# Autodesk Inventor assembly: Full_model
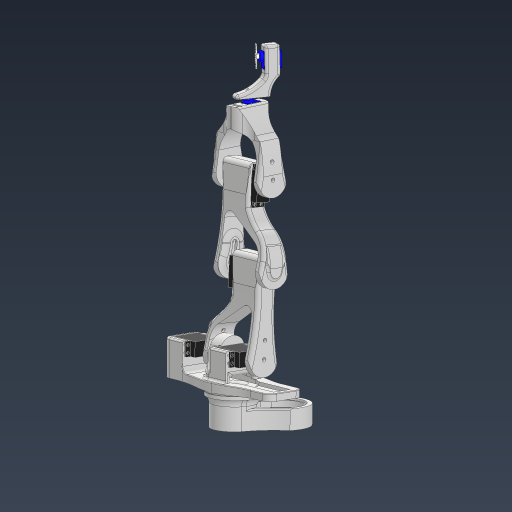
[picture p0: Inventor's stored thumbnail of the model, 512x512]
Saved by Autodesk Inventor 2024 (Build 280153000, 153)
## iProperties
Created: 2025-08-29
Part Number: Full_model
Document SubType Name: Assembly
Designer: Piter
Author: Piter
## Documents named in this file (9)
- C:\Users\Piter\OneDrive\Pulpit\Robots\david_Arm\Davie-Robot-Arm\3D Models\Full_model.iam
- C:\Users\Piter\OneDrive\Pulpit\Robots\david_Arm\Davie-Robot-Arm\3D Models\Arm2.ipt
- C:\Users\Piter\OneDrive\Pulpit\Robots\david_Arm\Davie-Robot-Arm\3D Models\feetech_25kg_servo.ipt
- C:\Users\Piter\OneDrive\Pulpit\Robots\david_Arm\Davie-Robot-Arm\3D Models\Arm3.ipt
- C:\Users\Piter\OneDrive\Pulpit\Robots\david_Arm\Davie-Robot-Arm\3D Models\TowerPro SG90 M.ipt
- C:\Users\Piter\OneDrive\Pulpit\Robots\david_Arm\Davie-Robot-Arm\3D Models\Arm4.ipt
- C:\Users\Piter\OneDrive\Pulpit\Robots\david_Arm\Davie-Robot-Arm\3D Models\Arm2_2SERVO.ipt
- C:\Users\Piter\OneDrive\Pulpit\Robots\david_Arm\Davie-Robot-Arm\3D Models\Base_v3_test.ipt
- C:\Users\Piter\OneDrive\Pulpit\Robots\david_Arm\Davie-Robot-Arm\3D Models\Axis1_v2.ipt
## Components (12 placed, 8 different names)
1. Arm2:1 — Rotational:4, Rotational:6, Rigid:7
2. feetech_25kg_servo:1 — Rigid:6
3. Arm3:1 — Rotational:4, Rigid:1
4. TowerPro SG90 M:1 — Rigid:1, Rotational:5
5. Arm4:1 — Rotational:5, Rigid:5
6. TowerPro SG90 M:2 — Rigid:5
7. Arm2_2SERVO:1 — Rigid:6, Rotational:6, Rotational:8
8. feetech_25kg_servo:2 — Rigid:7
9. feetech_25kg_servo:3 — Rigid:9
10. feetech_25kg_servo:4 — Rigid:8
11. Axis1_v2:1 — Rigid:8, Rigid:9, Rotational:8, Rotational:9
12. Base_v3_test:1 — Rotational:9
## Relationships (11: WeldJoint 6, RevoluteJoint 5)
- Rotational:4 [RevoluteJoint]: Arm2:1 ↔ Arm3:1
- Rigid:1 [WeldJoint]: Arm3:1 ↔ TowerPro SG90 M:1
- Rotational:5 [RevoluteJoint]: TowerPro SG90 M:1 ↔ Arm4:1
- Rigid:5 [WeldJoint]: Arm4:1 ↔ TowerPro SG90 M:2
- Rigid:6 [WeldJoint]: feetech_25kg_servo:1 ↔ Arm2_2SERVO:1
- Rotational:6 [RevoluteJoint]: Arm2:1 ↔ Arm2_2SERVO:1
- Rigid:7 [WeldJoint]: Arm2:1 ↔ feetech_25kg_servo:2
- Rigid:8 [WeldJoint]: feetech_25kg_servo:4 ↔ Axis1_v2:1
- Rigid:9 [WeldJoint]: feetech_25kg_servo:3 ↔ Axis1_v2:1
- Rotational:8 [RevoluteJoint]: Arm2_2SERVO:1 ↔ Axis1_v2:1
- Rotational:9 [RevoluteJoint]: Axis1_v2:1 ↔ Base_v3_test:1
